# Autodesk Inventor assembly: suport tija
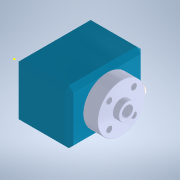
[picture p0: Inventor's stored thumbnail of the model, 180x180]
Saved by Autodesk Inventor 2022 (Build 260153000, 153)
## iProperties
Created: 2022-03-04
Part Number: suport tija
Document SubType Name: Assembly
Designer: Oana
Author: Oana
## Documents named in this file (3)
- D:\salvari\aplicatii-proiecte\infoeducatia 2022\proiectare\pat_scanare\suport tija.iam
- D:\salvari\aplicatii-proiecte\infoeducatia 2022\proiectare\pat_scanare\suport tija.ipt
- D:\salvari\aplicatii-proiecte\infoeducatia 2022\proiectare\piese\39172_txm-axle hub with set screw (1).ipt
## Components (2 placed, 2 different names)
1. suport tija:1 — Rotational:1
2. 39172_txm-axle hub with set screw (1):1 — Rotational:1
## Relationships (1: RevoluteJoint 1)
- Rotational:1 [RevoluteJoint]: suport tija:1 ↔ 39172_txm-axle hub with set screw (1):1
